# Autodesk Inventor assembly: 28아이들러_MIR
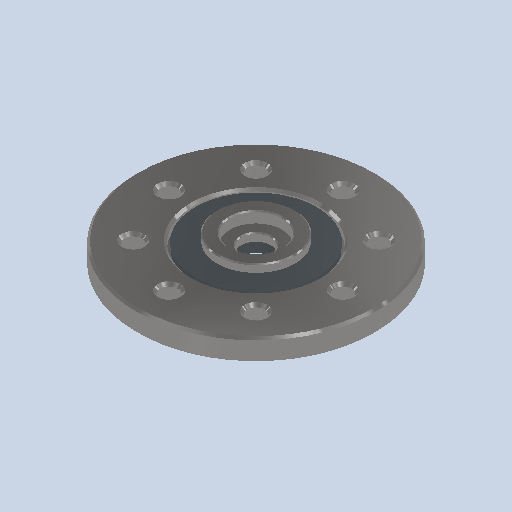
[picture p0: Inventor's stored thumbnail of the model, 512x512]
Saved by Autodesk Inventor 2024.3 (Build 283343000, 343)
## iProperties
Created: 2022-08-09
Part Number: 28아이들러_MIR
Document SubType Name: Assembly
Designer: 구지현
Mass: 3 g
Surface Area: 13.0954 cm^2
Volume: 0.790597 cm^3
Author: 박지훈
## Documents named in this file (4)
- C:\Users\구지현\Documents\카카오톡 받은 파일\Hardware\ROBOTIS(Inventor 2024 ver.)\아이들러\28아이들러_MIR.iam
- C:\Users\구지현\Documents\카카오톡 받은 파일\Hardware\ROBOTIS(Inventor 2024 ver.)\아이들러\MF106ZZ_MIR.ipt
- C:\Users\구지현\Documents\카카오톡 받은 파일\Hardware\ROBOTIS(Inventor 2024 ver.)\아이들러\RX28-CAP_MIR.ipt
- C:\Users\구지현\Documents\카카오톡 받은 파일\Hardware\ROBOTIS(Inventor 2024 ver.)\아이들러\HN07-i101_MIR.ipt
## Components (3 placed, 3 different names)
1. MF106ZZ_MIR:1 — 삽입:2, 삽입:3
2. RX28-CAP_MIR:1 — 삽입:2
3. HN07-i101_MIR:1 — 삽입:3
## Relationships (2: Insert 2)
- 삽입:2 [Insert]: MF106ZZ_MIR:1 ↔ RX28-CAP_MIR:1
- 삽입:3 [Insert]: MF106ZZ_MIR:1 ↔ HN07-i101_MIR:1
